# Autodesk Inventor assembly: myPalletizer_230708
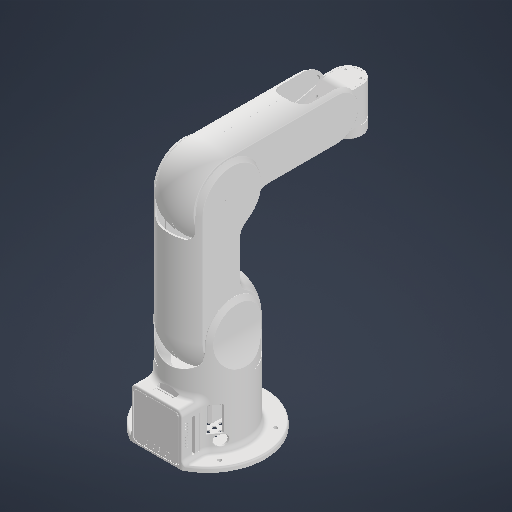
[picture p0: Inventor's stored thumbnail of the model, 512x512]
Saved by Autodesk Inventor 2026.2 (Build 302298000, 298)
## iProperties
Created: 2021-09-28
Part Number: myPalletizer_230708
Document SubType Name: Assembly
Designer: nicoa
Title: MYPALLETIZER_ASM
Author: Admin
Revision Number: 228LAST_VERSION
Sending System: CREO PARAMETRIC BY PTC INC, 2017380
Preprocessor: CREO PARAMETRIC BY PTC INC, 2017380
## Documents named in this file (7)
- C:\Users\nicoa\Desktop\Universidad\ERP\preERP\mechanical\step\myPalletizer_230708\myPalletizer_230708\myPalletizer_230708.iam
- C:\Users\nicoa\Desktop\Universidad\ERP\preERP\mechanical\step\base.iam
- C:\Users\nicoa\Desktop\Universidad\ERP\preERP\mechanical\step\rot.iam
- C:\Users\nicoa\Desktop\Universidad\ERP\preERP\mechanical\step\linkone.iam
- C:\Users\nicoa\Desktop\Universidad\ERP\preERP\mechanical\step\link2.iam
- C:\Users\nicoa\Desktop\Universidad\ERP\preERP\mechanical\step\act1.iam
- C:\Users\nicoa\Desktop\Universidad\ERP\preERP\mechanical\step\act2.iam
## Components (6 placed, 6 different names)
1. base:1 [sub-assembly] — rotation
2. rot:1 [sub-assembly] — rotation, Rotational:2
3. linkone:1 [sub-assembly] — Rotational:2, Rotational:3
4. link2:1 [sub-assembly] — Rotational:3
5. act1:1 [sub-assembly]
6. act2:1 [sub-assembly]
## Relationships (3: RevoluteJoint 3)
- rotation [RevoluteJoint]: base:1 ↔ rot:1
- Rotational:2 [RevoluteJoint] (1.25 mm): rot:1 ↔ linkone:1
- Rotational:3 [RevoluteJoint] (1.25 mm): linkone:1 ↔ link2:1
